# Autodesk Inventor assembly: ScannerMountingOption2
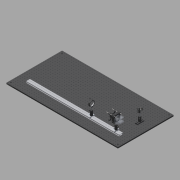
[picture p0: Inventor's stored thumbnail of the model, 180x180]
Saved by Autodesk Inventor 2018 (Build 220112000, 112)
## iProperties
Created: 2018-09-17
Part Number: ScannerMountingOption2
Document SubType Name: Assembly
Designer: Robert Campbell
Author: Robert Campbell
## Documents named in this file (9)
- X:\home\work\Documents\MF_BenchOptics\CAD_files\ScannerMountingOption2.iam
- X:\home\work\Documents\MF_BenchOptics\CAD_files\MB60120_M-Solidworks.ipt
- X:\home\work\Documents\MF_BenchOptics\CAD_files\XT66DP-1000-Solidworks.ipt
- X:\home\work\Documents\MF_BenchOptics\CAD_files\first_mirror.iam
- X:\home\work\Documents\MF_BenchOptics\CAD_files\MountedScanners.iam
- W:\home\work\Documents\MF_BenchOptics\CAD_files\ER4-Solidworks.ipt
- W:\home\work\Documents\MF_BenchOptics\CAD_files\LCP02_M-Solidworks.ipt
- W:\home\work\Documents\MF_BenchOptics\CAD_files\SM1L10-Solidworks.ipt
- W:\home\work\Documents\MF_BenchOptics\CAD_files\LM2_lensholder_on_mount.iam
## Components (9 placed, 8 different names)
1. MB60120_M-Solidworks:1 — Mate:1, Mate:21
2. XT66DP-1000-Solidworks:1 — Mate:1, Angle:1, Mate:22, Mate:28, Angle:3
3. first_mirror:1 [sub-assembly] — Mate:21
4. MountedScanners:1 [sub-assembly] — Angle:1, Mate:22, Mate:23, Angle:2, Mate:24, Mate:25
5. ER4-Solidworks:1 — Mate:24
6. ER4-Solidworks:2 — Mate:25
7. LCP02_M-Solidworks:1 — Mate:23, Angle:2, Mate:26, Mate:27
8. SM1L10-Solidworks:1 — Mate:26, Mate:27
9. LM2_lensholder_on_mount:1 [sub-assembly] — Mate:28, Angle:3
## Relationships (12: Mate 9, Angle 3)
- Mate:1: MB60120_M-Solidworks:1 ↔ XT66DP-1000-Solidworks:1
- Mate:21: MB60120_M-Solidworks:1 ↔ first_mirror:1
- Angle:1 (0 deg): XT66DP-1000-Solidworks:1 ↔ MountedScanners:1
- Mate:22: XT66DP-1000-Solidworks:1 ↔ MountedScanners:1
- Mate:23: MountedScanners:1 ↔ LCP02_M-Solidworks:1
- Angle:2 (0 deg): MountedScanners:1 ↔ LCP02_M-Solidworks:1
- Mate:24: MountedScanners:1 ↔ ER4-Solidworks:1
- Mate:25: MountedScanners:1 ↔ ER4-Solidworks:2
- Mate:26: LCP02_M-Solidworks:1 ↔ SM1L10-Solidworks:1
- Mate:27: LCP02_M-Solidworks:1 ↔ SM1L10-Solidworks:1
- Mate:28: XT66DP-1000-Solidworks:1 ↔ LM2_lensholder_on_mount:1
- Angle:3 (0 deg): XT66DP-1000-Solidworks:1 ↔ LM2_lensholder_on_mount:1
